# Autodesk Inventor assembly: medium
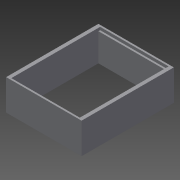
[picture p0: Inventor's stored thumbnail of the model, 180x180]
Saved by Autodesk Inventor 2014 SP1 (Build 180222100, 222)
## iProperties
Created: 2014-02-23
Part Number: medium
Document SubType Name: Assembly
Designer: Chris
Mass: 5525.26 g
Surface Area: 7084.66 cm^2
Volume: 5525.26 cm^3
Density: 1 g/cm^3
Author: Chris
## Documents named in this file (3)
- C:\Users\Chris\Documents\projects\langstroth_plain\medium\medium.iam
- C:\Users\Chris\Documents\projects\langstroth_plain\medium\medium_end.ipt
- C:\Users\Chris\Documents\projects\langstroth_plain\medium\medium_side.ipt
## Components (4 placed, 2 different names)
1. medium_end:1 — Flush:1, Flush:3, Flush:5, Flush:6, Flush:7, Flush:8
2. medium_end:2 — Flush:9, Flush:10, Flush:11
3. medium_side:1 — Flush:6, Flush:7, Flush:8
4. medium_side:2 — Flush:1, Flush:3, Flush:5, Flush:9, Flush:10, Flush:11
## Relationships (9: Flush 9)
- Flush:1: medium_end:1 ↔ medium_side:2
- Flush:3: medium_end:1 ↔ medium_side:2
- Flush:5: medium_end:1 ↔ medium_side:2
- Flush:6: medium_end:1 ↔ medium_side:1
- Flush:7: medium_end:1 ↔ medium_side:1
- Flush:8: medium_end:1 ↔ medium_side:1
- Flush:9: medium_end:2 ↔ medium_side:2
- Flush:10: medium_end:2 ↔ medium_side:2
- Flush:11: medium_end:2 ↔ medium_side:2
